# Autodesk Inventor assembly: КВ33.044.100 - Механизм перемещения захвата
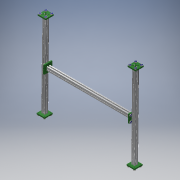
[picture p0: Inventor's stored thumbnail of the model, 180x180]
Saved by Autodesk Inventor 2019 (Build 230136000, 136)
## iProperties
Created: 2019-07-21
Part Number: КВ33.044.100 - Механизм перемещения захвата
Material: Типовые
Document SubType Name: Assembly
Designer: Петров Иван
Author: Петров Иван
## Documents named in this file (3)
- E:\IVAN\Kvantoriada2019\optimal_gripper\hardware\КВ33.044.100 - Механизм перемещения захвата.iam
- E:\IVAN\Kvantoriada2019\optimal_gripper\hardware\Стандартные изделия\Профиль станочный 30x30x720.ipt
- E:\IVAN\Kvantoriada2019\optimal_gripper\hardware\КВ33.044.200 - Каретка оси Х.iam
## Components (9 placed, 2 different names)
1. Профиль станочный 30x30x720:1 — Совмещение:1, Совмещение:2, Совмещение:3, Совмещение:4, Совмещение:5, Совмещение:6, Совмещение:13, Касательность:1, Касательность:2
2. КВ33.044.200 - Каретка оси Х:1 [sub-assembly] — Совмещение:1, Совмещение:2, Совмещение:3
3. КВ33.044.200 - Каретка оси Х:2 [sub-assembly] — Совмещение:4, Совмещение:5, Совмещение:6
4. Профиль станочный 30x30x720:2 — Совмещение:7, Совмещение:8, Совмещение:9, Совмещение:10, Совмещение:11, Совмещение:12, Совмещение:14, Касательность:3, Касательность:4
5. КВ33.044.200 - Каретка оси Х:3 [sub-assembly] — Совмещение:7, Совмещение:8, Совмещение:9
6. КВ33.044.200 - Каретка оси Х:4 [sub-assembly] — Совмещение:10, Совмещение:11, Совмещение:12
7. КВ33.044.200 - Каретка оси Х:5 [sub-assembly] — Совмещение:13, Касательность:1, Касательность:2, Совмещение:19, Совмещение:20, Совмещение:21
8. КВ33.044.200 - Каретка оси Х:6 [sub-assembly] — Совмещение:14, Касательность:3, Касательность:4, Совмещение:15, Совмещение:16, Совмещение:17
9. Профиль станочный 30x30x720:3 — Совмещение:15, Совмещение:16, Совмещение:17, Совмещение:19, Совмещение:20, Совмещение:21
## Relationships (24: Mate 20, Tangent 4)
- Совмещение:1 [Mate]: Профиль станочный 30x30x720:1 ↔ КВ33.044.200 - Каретка оси Х:1
- Совмещение:2 [Mate]: Профиль станочный 30x30x720:1 ↔ КВ33.044.200 - Каретка оси Х:1
- Совмещение:3 [Mate]: Профиль станочный 30x30x720:1 ↔ КВ33.044.200 - Каретка оси Х:1
- Совмещение:4 [Mate]: Профиль станочный 30x30x720:1 ↔ КВ33.044.200 - Каретка оси Х:2
- Совмещение:5 [Mate]: Профиль станочный 30x30x720:1 ↔ КВ33.044.200 - Каретка оси Х:2
- Совмещение:6 [Mate]: Профиль станочный 30x30x720:1 ↔ КВ33.044.200 - Каретка оси Х:2
- Совмещение:7 [Mate]: Профиль станочный 30x30x720:2 ↔ КВ33.044.200 - Каретка оси Х:3
- Совмещение:8 [Mate]: Профиль станочный 30x30x720:2 ↔ КВ33.044.200 - Каретка оси Х:3
- Совмещение:9 [Mate]: Профиль станочный 30x30x720:2 ↔ КВ33.044.200 - Каретка оси Х:3
- Совмещение:10 [Mate]: Профиль станочный 30x30x720:2 ↔ КВ33.044.200 - Каретка оси Х:4
- Совмещение:11 [Mate]: Профиль станочный 30x30x720:2 ↔ КВ33.044.200 - Каретка оси Х:4
- Совмещение:12 [Mate]: Профиль станочный 30x30x720:2 ↔ КВ33.044.200 - Каретка оси Х:4
- Совмещение:13 [Mate] (1.5 mm): Профиль станочный 30x30x720:1 ↔ КВ33.044.200 - Каретка оси Х:5
- Касательность:1 [Tangent]: Профиль станочный 30x30x720:1 ↔ КВ33.044.200 - Каретка оси Х:5
- Касательность:2 [Tangent]: Профиль станочный 30x30x720:1 ↔ КВ33.044.200 - Каретка оси Х:5
- Совмещение:14 [Mate] (1.5 mm): Профиль станочный 30x30x720:2 ↔ КВ33.044.200 - Каретка оси Х:6
- Касательность:3 [Tangent]: Профиль станочный 30x30x720:2 ↔ КВ33.044.200 - Каретка оси Х:6
- Касательность:4 [Tangent]: Профиль станочный 30x30x720:2 ↔ КВ33.044.200 - Каретка оси Х:6
- Совмещение:15 [Mate]: КВ33.044.200 - Каретка оси Х:6 ↔ Профиль станочный 30x30x720:3
- Совмещение:16 [Mate]: КВ33.044.200 - Каретка оси Х:6 ↔ Профиль станочный 30x30x720:3
- Совмещение:17 [Mate]: КВ33.044.200 - Каретка оси Х:6 ↔ Профиль станочный 30x30x720:3
- Совмещение:19 [Mate]: КВ33.044.200 - Каретка оси Х:5 ↔ Профиль станочный 30x30x720:3
- Совмещение:20 [Mate]: КВ33.044.200 - Каретка оси Х:5 ↔ Профиль станочный 30x30x720:3
- Совмещение:21 [Mate]: КВ33.044.200 - Каретка оси Х:5 ↔ Профиль станочный 30x30x720:3
